# Autodesk Inventor assembly: 2AM-17-A-3200 - wheels for outside slider
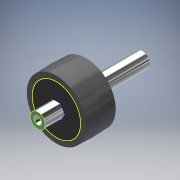
[picture p0: Inventor's stored thumbnail of the model, 180x180]
Saved by Autodesk Inventor 2017 (Build 210142000, 142)
## iProperties
Created: 2017-12-27
Part Number: 2AM-17-A-3200 - wheels for outside slider
Document SubType Name: Assembly
Designer: Micah
Mass: 66.5842 g
Surface Area: 269.788 cm^2
Volume: 47.251 cm^3
Density: 1.40916 g/cm^3
Author: Micah
## Documents named in this file (5)
- C:\Users\Micah\Desktop\inventor\CADathon-2017\2AM-17-A-0200 - Smokestack Elevator\2AM-17-A-3200 - wheels for outside slider.iam
- C:\Users\Micah\Desktop\inventor\CADathon-2017\2AM-17-A-0200 - Smokestack Elevator\COTS\2in Wheel Intergrated 0500 HEX Hub.ipt
- C:\Users\Micah\Desktop\inventor\CADathon-2017\2AM-17-A-0200 - Smokestack Elevator\2AM-17-P-3201 - hex to tube adapter.ipt
- C:\Users\Micah\Desktop\inventor\CADathon-2017\2AM-17-A-0200 - Smokestack Elevator\COTS\2in Tread.ipt
- C:\Users\Micah\Desktop\inventor\CADathon-2017\2AM-17-A-0200 - Smokestack Elevator\2AM-17-P-3202 - tube shaft.ipt
## Components (4 placed, 4 different names)
1. 2in Wheel Intergrated 0500 HEX Hub:1
2. 2AM-17-P-3201 - hex to tube adapter:1 — Rigid:2
3. 2in Tread:1
4. 2AM-17-P-3202 - tube shaft:1 — Rigid:2
## Relationships (3: WeldJoint 2, RevoluteJoint 1)
- [WeldJoint]: 2in Wheel Intergrated 0500 HEX Hub:1 ↔ 2AM-17-P-3201 - hex to tube adapter:1
- [RevoluteJoint]: 2in Wheel Intergrated 0500 HEX Hub:1 ↔ 2in Tread:1
- Rigid:2 [WeldJoint] (47.625 mm): 2AM-17-P-3201 - hex to tube adapter:1 ↔ 2AM-17-P-3202 - tube shaft:1
## Named parameters: d0_d2 = 0 mm
